# Autodesk Inventor assembly: TümSistem
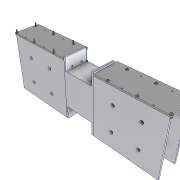
[picture p0: Inventor's stored thumbnail of the model, 180x180]
Saved by Autodesk Inventor 2020.3 (Build 243373000, 373)
## iProperties
Created: 2020-12-04
Part Number: TümSistem
Document SubType Name: Assembly
Designer: Yusuf
Mass: 2701.27 g
Surface Area: 8527.94 cm^2
Volume: 2632.53 cm^3
Density: 1.02611 g/cm^3
Author: Yusuf
## Documents named in this file (7)
- C:\Users\Yusuf\Desktop\SunCollector_Autodesk\TümSistem.iam
- C:\Users\Yusuf\Desktop\SunCollector_Autodesk\MiddlePart.ipt
- C:\Users\Yusuf\Desktop\SunCollector_Autodesk\SunTrackerHolder.ipt
- C:\Users\Yusuf\Desktop\SunCollector_Autodesk\MiddleGlass.ipt
- C:\Users\Yusuf\Desktop\SunCollector_Autodesk\PCB.ipt
- C:\Users\Yusuf\Desktop\SunCollector_Autodesk\ÜstKısım.iam
- C:\Users\Yusuf\Desktop\SunCollector_Autodesk\ÜstKısım_MirrorV2.iam
## Components (6 placed, 6 different names)
1. MiddlePart:1 — Mate:1, Mate:2, Flush:2, Mate:3, Flush:3, Angle:1, Mate:4, Mate:5, Mate:6, Mate:7, Flush:4, Flush:5
2. SunTrackerHolder:1 — Mate:1, Flush:3, Angle:1
3. MiddleGlass:1 — Mate:2, Flush:2, Mate:3
4. PCB:1 — Mate:4, Mate:5, Mate:6
5. ÜstKısım:1 [sub-assembly] — Mate:7, Flush:4, Flush:5
6. ÜstKısım_MirrorV2:1 [sub-assembly]
## Relationships (12: Mate 7, Flush 4, Angle 1)
- Mate:1: MiddlePart:1 ↔ SunTrackerHolder:1
- Mate:2: MiddlePart:1 ↔ MiddleGlass:1
- Flush:2: MiddlePart:1 ↔ MiddleGlass:1
- Mate:3: MiddlePart:1 ↔ MiddleGlass:1
- Flush:3 (3 mm): MiddlePart:1 ↔ SunTrackerHolder:1
- Angle:1 (0 deg): MiddlePart:1 ↔ SunTrackerHolder:1
- Mate:4 (2 mm): MiddlePart:1 ↔ PCB:1
- Mate:5: MiddlePart:1 ↔ PCB:1
- Mate:6 (1 mm): MiddlePart:1 ↔ PCB:1
- Mate:7: MiddlePart:1 ↔ ÜstKısım:1
- Flush:4: MiddlePart:1 ↔ ÜstKısım:1
- Flush:5: MiddlePart:1 ↔ ÜstKısım:1
